# Autodesk Inventor assembly: ObjektivmountGesamt
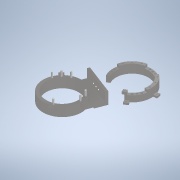
[picture p0: Inventor's stored thumbnail of the model, 180x180]
Saved by Autodesk Inventor 2021 (Build 250183000, 183)
## iProperties
Created: 2021-01-15
Part Number: ObjektivmountGesamt
Document SubType Name: Assembly
Designer: Paul
Mass: 1167.02 g
Surface Area: 1432.91 cm^2
Volume: 335.631 cm^3
Density: 3.4771 g/cm^3
Author: Paul
## Documents named in this file (7)
- E:\Data\Daniel\Setup\Objektivmount\ObjektivmountGesamt.iam
- E:\Data\Daniel\Setup\Objektivmount\Objektivmount01.ipt
- E:\Data\Daniel\Setup\Objektivmount\ObererMount01.ipt
- E:\Data\Daniel\Setup\Objektivmount\AGATHON_N6500ZylindrischMiniatur6500003030(1)\N6500 Zylindrisch Miniatur 6500_003_030.ipt
- E:\Data\Daniel\Setup\Objektivmount\AGATHON_N7650KugelkaefigausMessingMiniatur7650003015(1)\N7650 Kugelkaefig aus Messing Miniatur 7650_003_015.ipt
- C:\Users\Paul\Desktop\Newport-LP-2A.ipt
- E:\Data\Daniel\Setup\Objektivmount\AGATHON_N7800BuchsemitKleberille7800004015\N7800 Buchse mit Kleberille 7800_004_015.ipt
## Components (21 placed, 6 different names)
1. Objektivmount01:1 — Einfügen:12, Einfügen:13, Einfügen:14, Einfügen:15, Einfügen:16, Einfügen:22
2. ObererMount01:1 — Einfügen:17, Einfügen:18, Einfügen:19, Einfügen:20, Einfügen:21, Einfügen:24
3. N6500 Zylindrisch Miniatur 6500_003_030:1 — Einfügen:11
4. N6500 Zylindrisch Miniatur 6500_003_030:2 — Einfügen:7
5. N6500 Zylindrisch Miniatur 6500_003_030:3 — Einfügen:8
6. N7650 Kugelkaefig aus Messing Miniatur 7650_003_015:1 — Einfügen:7, Einfügen:19
7. N7650 Kugelkaefig aus Messing Miniatur 7650_003_015:2 — Einfügen:8, Einfügen:18
8. N7650 Kugelkaefig aus Messing Miniatur 7650_003_015:3 — Einfügen:9, Einfügen:21
9. N6500 Zylindrisch Miniatur 6500_003_030:4 — Einfügen:9
10. N6500 Zylindrisch Miniatur 6500_003_030:5 — Einfügen:10
11. N7650 Kugelkaefig aus Messing Miniatur 7650_003_015:4 — Einfügen:10, Einfügen:20
12. N7650 Kugelkaefig aus Messing Miniatur 7650_003_015:5 — Einfügen:11, Einfügen:17
13. Newport-LP-2A:1
14. N7800 Buchse mit Kleberille 7800_004_015:1 — Einfügen:12
15. N7800 Buchse mit Kleberille 7800_004_015:2 — Einfügen:13
16. N7800 Buchse mit Kleberille 7800_004_015:3 — Einfügen:14
17. N7800 Buchse mit Kleberille 7800_004_015:4 — Einfügen:15
18. N7800 Buchse mit Kleberille 7800_004_015:5 — Einfügen:16
19. N7800 Buchse mit Kleberille 7800_004_015:6 — Einfügen:22
20. N6500 Zylindrisch Miniatur 6500_003_030:6
21. N7650 Kugelkaefig aus Messing Miniatur 7650_003_015:6 — Einfügen:24
## Relationships (18: Insert 18)
- Einfügen:7 [Insert]: N6500 Zylindrisch Miniatur 6500_003_030:2 ↔ N7650 Kugelkaefig aus Messing Miniatur 7650_003_015:1
- Einfügen:8 [Insert]: N6500 Zylindrisch Miniatur 6500_003_030:3 ↔ N7650 Kugelkaefig aus Messing Miniatur 7650_003_015:2
- Einfügen:9 [Insert]: N7650 Kugelkaefig aus Messing Miniatur 7650_003_015:3 ↔ N6500 Zylindrisch Miniatur 6500_003_030:4
- Einfügen:10 [Insert]: N6500 Zylindrisch Miniatur 6500_003_030:5 ↔ N7650 Kugelkaefig aus Messing Miniatur 7650_003_015:4
- Einfügen:11 [Insert]: N6500 Zylindrisch Miniatur 6500_003_030:1 ↔ N7650 Kugelkaefig aus Messing Miniatur 7650_003_015:5
- Einfügen:12 [Insert]: Objektivmount01:1 ↔ N7800 Buchse mit Kleberille 7800_004_015:1
- Einfügen:13 [Insert]: Objektivmount01:1 ↔ N7800 Buchse mit Kleberille 7800_004_015:2
- Einfügen:14 [Insert]: Objektivmount01:1 ↔ N7800 Buchse mit Kleberille 7800_004_015:3
- Einfügen:15 [Insert]: Objektivmount01:1 ↔ N7800 Buchse mit Kleberille 7800_004_015:4
- Einfügen:16 [Insert]: Objektivmount01:1 ↔ N7800 Buchse mit Kleberille 7800_004_015:5
- Einfügen:17 [Insert]: ObererMount01:1 ↔ N7650 Kugelkaefig aus Messing Miniatur 7650_003_015:5
- Einfügen:18 [Insert]: ObererMount01:1 ↔ N7650 Kugelkaefig aus Messing Miniatur 7650_003_015:2
- Einfügen:19 [Insert]: ObererMount01:1 ↔ N7650 Kugelkaefig aus Messing Miniatur 7650_003_015:1
- Einfügen:20 [Insert]: ObererMount01:1 ↔ N7650 Kugelkaefig aus Messing Miniatur 7650_003_015:4
- Einfügen:21 [Insert]: ObererMount01:1 ↔ N7650 Kugelkaefig aus Messing Miniatur 7650_003_015:3
- Einfügen:22 [Insert]: Objektivmount01:1 ↔ N7800 Buchse mit Kleberille 7800_004_015:6
- [Insert]: N6500 Zylindrisch Miniatur 6500_003_030:6 ↔ N7650 Kugelkaefig aus Messing Miniatur 7650_003_015:6
- Einfügen:24 [Insert]: ObererMount01:1 ↔ N7650 Kugelkaefig aus Messing Miniatur 7650_003_015:6
## Named parameters: Innenradius = 94 mm, Aussenradius = 112 mm, m3 = 3.5 mm, Stufenhöhe = 7 mm, RadiusLoecher = 104 mm, m3Kopf = 6 mm, MinimalabstandKuehlung = 7 mm, InnenradiusOberhalbSchrauben = 98 mm, ExtrusionOberhalbSchrauben = 5 mm, Plateaudurchmesser = 10 mm, Verbindung_d2 = 8 mm, Plateauhoehe = 18 mm, Verbindung_d1 = 3 mm, Verbindung_d2_tiefe = 15 mm, Verbindung_d1_tiefe = 15 mm, d44_d11 = 0 mm
